# Autodesk Inventor assembly: main body
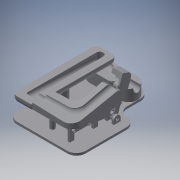
[picture p0: Inventor's stored thumbnail of the model, 180x180]
Saved by Autodesk Inventor 2016 (Build 200138000, 138)
## iProperties
Created: 2018-05-06
Part Number: main body
Material: 一般
Document SubType Name: Assembly
Designer: 黃胤瑋
Author: 黃胤瑋
## Documents named in this file (18)
- C:\Users\黃胤瑋\Desktop\mechanism\second generation\main body.iam
- C:\Users\黃胤瑋\Desktop\mechanism\second generation\實體1.ipt
- C:\Users\黃胤瑋\Desktop\mechanism\second generation\實體2.ipt
- C:\Users\黃胤瑋\Desktop\mechanism\second generation\實體3.ipt
- C:\Users\黃胤瑋\Desktop\mechanism\second generation\實體4.ipt
- C:\Users\黃胤瑋\Desktop\mechanism\second generation\實體5.ipt
- C:\Users\黃胤瑋\Desktop\mechanism\second generation\實體6.ipt
- C:\Users\黃胤瑋\Desktop\mechanism\second generation\實體7.ipt
- C:\Users\黃胤瑋\Desktop\mechanism\second generation\實體8.ipt
- C:\Users\黃胤瑋\Desktop\mechanism\second generation\實體9.ipt
- C:\Users\黃胤瑋\Desktop\mechanism\second generation\02連桿25.ipt
- C:\Users\黃胤瑋\Desktop\mechanism\second generation\03連桿15.ipt
- C:\Users\黃胤瑋\Desktop\mechanism\second generation\馬達.ipt
- C:\Users\黃胤瑋\Desktop\mechanism\second generation\實體10.ipt
- C:\Users\黃胤瑋\Desktop\mechanism\second generation\銷.ipt
- C:\Users\黃胤瑋\Documents\Inventor\Content Center Files\R2016\zh-TW\JIS B 1176\JIS B 1176 - M4 x 12.ipt
- C:\Users\黃胤瑋\Documents\Inventor\Content Center Files\R2016\zh-TW\JIS B 1176\JIS B 1176 - M4 x 16.ipt
- C:\Users\黃胤瑋\Documents\Inventor\Content Center Files\R2016\zh-TW\JIS B 1181 U\JIS B 1181 - B M4.ipt
## Components (28 placed, 17 different names)
1. 實體1:1 — 貼合:15, 貼合:16, 貼合:17, 貼合:18, 角度:3, 角度:4, 貼合:21, 齊平:5, 貼合:24, 角度:5, 角度:6, 貼合:25, 貼合:26, 貼合:30, 貼合:31, 貼合:32, 角度:7, 齊平:6, 齊平:7
2. 實體2:1 — 貼合:21, 齊平:5, 貼合:22, 貼合:23, 角度:5
3. 實體3:1 — 貼合:31, 貼合:32
4. 實體4:1 — 貼合:27, 貼合:28, 貼合:29
5. 實體5:1 — 貼合:15, 貼合:18, 角度:4, 貼合:28, 貼合:50, 貼合:51, 貼合:52, 貼合:53
6. 實體6:1 — 貼合:1, 貼合:2, 貼合:3, 貼合:16, 貼合:17, 角度:3, 貼合:43, 貼合:45
7. 實體7:1 — 貼合:24, 角度:6, 齊平:6
8. 實體8:1 — 貼合:25, 貼合:26, 貼合:27, 貼合:29
9. 實體9:1 — 貼合:30, 齊平:7
10. 02連桿25:1 — 貼合:5, 貼合:6, 貼合:9, 貼合:10, 貼合:33, 貼合:34, 貼合:58, 貼合:59
11. 03連桿15:1 — 貼合:4, 貼合:5, 貼合:6, 貼合:19, 角度:7, 貼合:61
12. 馬達:1 — 貼合:1, 貼合:2, 貼合:3, 貼合:4, 貼合:14, 齊平:4, 貼合:42, 貼合:44, 貼合:47, 貼合:49, 貼合:56, 貼合:57
13. 實體10:1 — 貼合:9, 貼合:10, 貼合:22, 貼合:23, 貼合:35, 貼合:36, 貼合:39, 貼合:41
14. 銷:4 — 貼合:14, 齊平:4, 貼合:19
15. JIS B 1176 - 公制 M4 x 12:2 — 貼合:33, 貼合:34, 貼合:40
16. JIS B 1176 - 公制 M4 x 16:1 — 貼合:35, 貼合:36, 貼合:37, 貼合:38
17. JIS B 1181 (無倒角) - 公制 B M4:1 — 貼合:37, 貼合:38, 貼合:39
18. JIS B 1181 (無倒角) - 公制 B M4:2 — 貼合:40, 貼合:41
19. JIS B 1176 - 公制 M4 x 12:3 — 貼合:42, 貼合:43, 貼合:48
20. JIS B 1176 - 公制 M4 x 12:4 — 貼合:44, 貼合:45, 貼合:46
21. JIS B 1181 (無倒角) - 公制 B M4:3 — 貼合:55, 貼合:57
22. JIS B 1181 (無倒角) - 公制 B M4:4 — 貼合:46, 貼合:47
23. JIS B 1181 (無倒角) - 公制 B M4:5 — 貼合:48, 貼合:49
24. JIS B 1181 (無倒角) - 公制 B M4:6 — 貼合:54, 貼合:56
25. JIS B 1176 - 公制 M4 x 12:5 — 貼合:51, 貼合:53, 貼合:55
26. JIS B 1176 - 公制 M4 x 12:6 — 貼合:50, 貼合:52, 貼合:54
27. JIS B 1176 - 公制 M4 x 12:7 — 貼合:58, 貼合:59, 貼合:60
28. JIS B 1181 (無倒角) - 公制 B M4:7 — 貼合:60, 貼合:61
## Relationships (64: Mate 55, Angle 5, Flush 4)
- 貼合:1 [Mate]: 實體6:1 ↔ 馬達:1
- 貼合:2 [Mate]: 實體6:1 ↔ 馬達:1
- 貼合:3 [Mate]: 實體6:1 ↔ 馬達:1
- 貼合:4 [Mate]: 03連桿15:1 ↔ 馬達:1
- 貼合:5 [Mate]: 02連桿25:1 ↔ 03連桿15:1
- 貼合:6 [Mate]: 02連桿25:1 ↔ 03連桿15:1
- 貼合:9 [Mate]: 02連桿25:1 ↔ 實體10:1
- 貼合:10 [Mate]: 02連桿25:1 ↔ 實體10:1
- 貼合:14 [Mate]: 馬達:1 ↔ 銷:4
- 齊平:4 [Flush]: 馬達:1 ↔ 銷:4
- 貼合:15 [Mate]: 實體1:1 ↔ 實體5:1
- 貼合:16 [Mate]: 實體1:1 ↔ 實體6:1
- 貼合:17 [Mate]: 實體1:1 ↔ 實體6:1
- 貼合:18 [Mate]: 實體1:1 ↔ 實體5:1
- 角度:3 [Angle] (0 deg): 實體1:1 ↔ 實體6:1
- 角度:4 [Angle] (0 deg): 實體1:1 ↔ 實體5:1
- 貼合:19 [Mate]: 03連桿15:1 ↔ 銷:4
- 貼合:21 [Mate]: 實體1:1 ↔ 實體2:1
- 齊平:5 [Flush]: 實體1:1 ↔ 實體2:1
- 貼合:22 [Mate]: 實體2:1 ↔ 實體10:1
- 貼合:23 [Mate]: 實體2:1 ↔ 實體10:1
- 貼合:24 [Mate]: 實體1:1 ↔ 實體7:1
- 角度:5 [Angle] (0 deg): 實體1:1 ↔ 實體2:1
- 角度:6 [Angle] (0 deg): 實體1:1 ↔ 實體7:1
- 貼合:25 [Mate]: 實體1:1 ↔ 實體8:1
- 貼合:26 [Mate]: 實體1:1 ↔ 實體8:1
- 貼合:27 [Mate]: 實體4:1 ↔ 實體8:1
- 貼合:28 [Mate]: 實體4:1 ↔ 實體5:1
- 貼合:29 [Mate]: 實體4:1 ↔ 實體8:1
- 貼合:30 [Mate]: 實體1:1 ↔ 實體9:1
- 貼合:31 [Mate]: 實體1:1 ↔ 實體3:1
- 貼合:32 [Mate]: 實體1:1 ↔ 實體3:1
- 角度:7 [Angle] (1238 deg): 實體1:1 ↔ 03連桿15:1
- 齊平:6 [Flush]: 實體1:1 ↔ 實體7:1
- 貼合:33 [Mate]: 02連桿25:1 ↔ JIS B 1176 - 公制 M4 x 12:2
- 貼合:34 [Mate]: 02連桿25:1 ↔ JIS B 1176 - 公制 M4 x 12:2
- 貼合:35 [Mate]: 實體10:1 ↔ JIS B 1176 - 公制 M4 x 16:1
- 貼合:36 [Mate]: 實體10:1 ↔ JIS B 1176 - 公制 M4 x 16:1
- 貼合:37 [Mate]: JIS B 1176 - 公制 M4 x 16:1 ↔ JIS B 1181 (無倒角) - 公制 B M4:1
- 貼合:38 [Mate]: JIS B 1176 - 公制 M4 x 16:1 ↔ JIS B 1181 (無倒角) - 公制 B M4:1
- 貼合:39 [Mate]: 實體10:1 ↔ JIS B 1181 (無倒角) - 公制 B M4:1
- 貼合:40 [Mate]: JIS B 1176 - 公制 M4 x 12:2 ↔ JIS B 1181 (無倒角) - 公制 B M4:2
- 貼合:41 [Mate]: 實體10:1 ↔ JIS B 1181 (無倒角) - 公制 B M4:2
- 貼合:42 [Mate]: 馬達:1 ↔ JIS B 1176 - 公制 M4 x 12:3
- 貼合:43 [Mate]: 實體6:1 ↔ JIS B 1176 - 公制 M4 x 12:3
- 貼合:44 [Mate]: 馬達:1 ↔ JIS B 1176 - 公制 M4 x 12:4
- 貼合:45 [Mate]: 實體6:1 ↔ JIS B 1176 - 公制 M4 x 12:4
- 貼合:46 [Mate]: JIS B 1176 - 公制 M4 x 12:4 ↔ JIS B 1181 (無倒角) - 公制 B M4:4
- 貼合:47 [Mate]: 馬達:1 ↔ JIS B 1181 (無倒角) - 公制 B M4:4
- 貼合:48 [Mate]: JIS B 1176 - 公制 M4 x 12:3 ↔ JIS B 1181 (無倒角) - 公制 B M4:5
- 貼合:49 [Mate]: 馬達:1 ↔ JIS B 1181 (無倒角) - 公制 B M4:5
- 貼合:50 [Mate]: 實體5:1 ↔ JIS B 1176 - 公制 M4 x 12:6
- 貼合:51 [Mate]: 實體5:1 ↔ JIS B 1176 - 公制 M4 x 12:5
- 貼合:52 [Mate]: 實體5:1 ↔ JIS B 1176 - 公制 M4 x 12:6
- 貼合:53 [Mate]: 實體5:1 ↔ JIS B 1176 - 公制 M4 x 12:5
- 貼合:54 [Mate]: JIS B 1181 (無倒角) - 公制 B M4:6 ↔ JIS B 1176 - 公制 M4 x 12:6
- 貼合:55 [Mate]: JIS B 1181 (無倒角) - 公制 B M4:3 ↔ JIS B 1176 - 公制 M4 x 12:5
- 貼合:56 [Mate]: 馬達:1 ↔ JIS B 1181 (無倒角) - 公制 B M4:6
- 貼合:57 [Mate]: 馬達:1 ↔ JIS B 1181 (無倒角) - 公制 B M4:3
- 貼合:58 [Mate]: 02連桿25:1 ↔ JIS B 1176 - 公制 M4 x 12:7
- 貼合:59 [Mate]: 02連桿25:1 ↔ JIS B 1176 - 公制 M4 x 12:7
- 貼合:60 [Mate]: JIS B 1176 - 公制 M4 x 12:7 ↔ JIS B 1181 (無倒角) - 公制 B M4:7
- 貼合:61 [Mate]: 03連桿15:1 ↔ JIS B 1181 (無倒角) - 公制 B M4:7
- 齊平:7 [Flush]: 實體1:1 ↔ 實體9:1
